# Autodesk Inventor assembly: AssemblyX
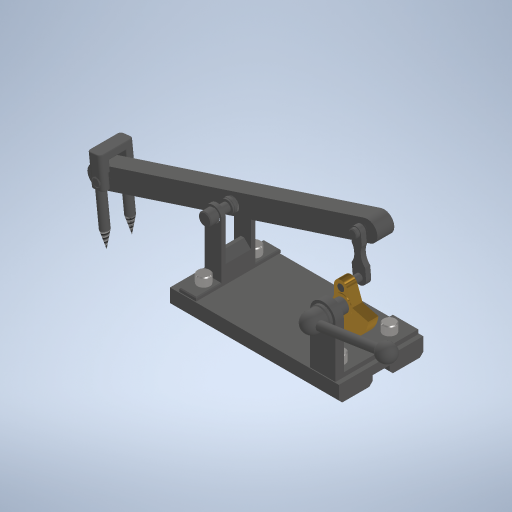
[picture p0: Inventor's stored thumbnail of the model, 512x512]
Saved by Autodesk Inventor 2023.2 (Build 272271000, 271)
## iProperties
Created: 2023-01-31
Part Number: AssemblyX
Document SubType Name: Assembly
Designer: Ayush
Author: Ayush
## Documents named in this file (13)
- F:\MS\SRH study\CAD projects\AssemblyX.iam
- F:\MS\SRH study\CAD projects\TAPPING MECHANISM TOOL Reference Moodle file\Groundplate.ipt
- F:\MS\SRH study\CAD projects\TAPPING MECHANISM TOOL Reference Moodle file\Rail stand.ipt
- F:\MS\SRH study\CAD projects\TAPPING MECHANISM TOOL Reference Moodle file\Half Bearing Block.ipt
- F:\MS\SRH study\CAD projects\TAPPING MECHANISM TOOL Reference Moodle file\Bearing Block.ipt
- F:\MS\SRH study\CAD projects\TAPPING MECHANISM TOOL Reference Moodle file\short bolt.ipt
- F:\MS\SRH study\CAD projects\TAPPING MECHANISM TOOL Reference Moodle file\KURBEL PART 8.ipt
- F:\MS\SRH study\CAD projects\TAPPING MECHANISM TOOL Reference Moodle file\KURBELZAPFEN NEW.ipt
- F:\MS\SRH study\CAD projects\TAPPING MECHANISM TOOL Reference Moodle file\PLEUEL short new.ipt
- F:\MS\SRH study\CAD projects\TAPPING MECHANISM TOOL Reference Moodle file\Lock pin.ipt
- F:\MS\SRH study\CAD projects\TAPPING MECHANISM TOOL Reference Moodle file\Lever.ipt
- F:\MS\SRH study\CAD projects\TAPPING MECHANISM TOOL Reference Moodle file\Bolt.ipt
- F:\MS\SRH study\CAD projects\TAPPING MECHANISM TOOL Reference Moodle file\Pin Marker.ipt
## Components (18 placed, 16 different names)
1. Groundplate:1 — Mate:1, Flush:1, Mate:2, Mate:3, Mate:4, Mate:5, Mate:6, Mate:7, Mate:8, Mate:9, Mate:10, Mate:11
2. Rail stand:1 — Mate:1, Flush:1, Mate:2
3. Rail stand:2 — Mate:3, Mate:4, Mate:5
4. Half Bearing Block:1 — Mate:6, Mate:7, Mate:8, Mate:12, Mate:13, Mate:36, Mate:37
5. Bearing Block:1 — Mate:9, Mate:10, Mate:11, Mate:27, Mate:28, Mate:34, Mate:35
6. short bolt:1 — Mate:12, Mate:13, Mate:14, Mate:15, Rotation:1
7. KURBEL PART 8:1 — Mate:14, Mate:15, Rotation:1, Mate:19, Mate:20
8. PLEUEL short new:1 — Mate:21, Mate:22, Mate:23, Mate:24, Mate:25
9. KURBELZAPFEN NEW:1 — Mate:19, Mate:20, Mate:21, Mate:22, Mate:23
10. Lock pin:1 — Mate:24, Mate:25, Flush:2, Mate:26
11. Lever:1 — Flush:2, Mate:26, Mate:29, Mate:30, Mate:31
12. Bolt:1 — Mate:27, Mate:28, Mate:29
13. Pin Marker:1 — Mate:32, Mate:33
14. Lock pin:2 — Mate:30, Mate:31, Mate:32, Mate:33
15. DIN 912 replaced by DIN EN ISO 4762 M4 * 12.1 — Mate:34
16. DIN 912 replaced by DIN EN ISO 4762 M4 * 12.2 — Mate:35
17. DIN 912 replaced by DIN EN ISO 4762 M4 * 12.3 — Mate:37
18. DIN 912 replaced by DIN EN ISO 4762 M4 * 12.4 — Mate:36
## Relationships (37: Mate 34, Flush 2, RelateRotation 1)
- Mate:1: Groundplate:1 ↔ Rail stand:1
- Flush:1: Groundplate:1 ↔ Rail stand:1
- Mate:2: Groundplate:1 ↔ Rail stand:1
- Mate:3: Groundplate:1 ↔ Rail stand:2
- Mate:4: Groundplate:1 ↔ Rail stand:2
- Mate:5: Groundplate:1 ↔ Rail stand:2
- Mate:6: Groundplate:1 ↔ Half Bearing Block:1
- Mate:7: Groundplate:1 ↔ Half Bearing Block:1
- Mate:8: Groundplate:1 ↔ Half Bearing Block:1
- Mate:9: Groundplate:1 ↔ Bearing Block:1
- Mate:10: Groundplate:1 ↔ Bearing Block:1
- Mate:11: Groundplate:1 ↔ Bearing Block:1
- Mate:12: Half Bearing Block:1 ↔ short bolt:1
- Mate:13: Half Bearing Block:1 ↔ short bolt:1
- Mate:14: short bolt:1 ↔ KURBEL PART 8:1
- Mate:15: short bolt:1 ↔ KURBEL PART 8:1
- Rotation:1 [RelateRotation] (1 ul): short bolt:1 ↔ KURBEL PART 8:1
- Mate:19: KURBEL PART 8:1 ↔ KURBELZAPFEN NEW:1
- Mate:20: KURBEL PART 8:1 ↔ KURBELZAPFEN NEW:1
- Mate:21: PLEUEL short new:1 ↔ KURBELZAPFEN NEW:1
- Mate:22: PLEUEL short new:1 ↔ KURBELZAPFEN NEW:1
- Mate:23: PLEUEL short new:1 ↔ KURBELZAPFEN NEW:1
- Mate:24: PLEUEL short new:1 ↔ Lock pin:1
- Mate:25: PLEUEL short new:1 ↔ Lock pin:1
- Flush:2: Lock pin:1 ↔ Lever:1
- Mate:26: Lock pin:1 ↔ Lever:1
- Mate:27: Bearing Block:1 ↔ Bolt:1
- Mate:28: Bearing Block:1 ↔ Bolt:1
- Mate:29: Lever:1 ↔ Bolt:1
- Mate:30: Lever:1 ↔ Lock pin:2
- Mate:31: Lever:1 ↔ Lock pin:2
- Mate:32: Pin Marker:1 ↔ Lock pin:2
- Mate:33: Pin Marker:1 ↔ Lock pin:2
- Mate:34: Bearing Block:1 ↔ DIN 912 replaced by DIN EN ISO 4762 M4 * 12.1
- Mate:35: Bearing Block:1 ↔ DIN 912 replaced by DIN EN ISO 4762 M4 * 12.2
- Mate:36: Half Bearing Block:1 ↔ DIN 912 replaced by DIN EN ISO 4762 M4 * 12.4
- Mate:37: Half Bearing Block:1 ↔ DIN 912 replaced by DIN EN ISO 4762 M4 * 12.3
